# Autodesk Inventor assembly: Battery Pack - Samsung 25R - 2xRows
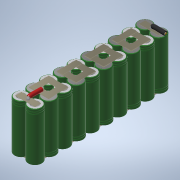
[picture p0: Inventor's stored thumbnail of the model, 180x180]
Saved by Autodesk Inventor 2020.1 (Build 241239000, 239)
## iProperties
Created: 2019-07-13
Part Number: Battery Pack - Samsung 25R - 2xRows
Document SubType Name: Assembly
Designer: Petar
Author: Petar
## Documents named in this file (5)
- D:\OMG\E-Board\CAD\Inventor\Electrical Components\Battery Pack\Samsung 25R\Battery Pack - Samsung 25R - 2xRows.iam
- D:\OMG\E-Board\CAD\Inventor\Electrical Components\Battery Pack\Samsung 25R\Battery Cell - Samsung.ipt
- D:\OMG\E-Board\CAD\Inventor\Electrical Components\Battery Pack\Samsung 25R\Nickel Strip.ipt
- D:\OMG\E-Board\CAD\Inventor\Electrical Components\Battery Pack\Samsung 25R\Solder (Plus).ipt
- D:\OMG\E-Board\CAD\Inventor\Electrical Components\Battery Pack\Samsung 25R\Solder (Minus).ipt
## Components (60 placed, 4 different names)
1. Battery Cell - Samsung:1 — Flush:1, Tangent:1, Flush:2, Flush:5, Flush:6, Tangent:3, Mate:6, Tangent:20, Tangent:22
2. Battery Cell - Samsung:2 — Flush:1, Tangent:1, Flush:2, Tangent:21
3. Battery Cell - Samsung:3 — Flush:5, Flush:6, Tangent:3, Flush:13, Tangent:7, Flush:14
4. Battery Cell - Samsung:4
5. Battery Cell - Samsung:5 — Flush:13, Tangent:7, Flush:14
6. Battery Cell - Samsung:6
7. Battery Cell - Samsung:7 — Flush:29, Tangent:15, Flush:30
8. Battery Cell - Samsung:8
9. Battery Cell - Samsung:9 — Flush:29, Tangent:15, Flush:30
10. Battery Cell - Samsung:10
11. Battery Cell - Samsung:11
12. Battery Cell - Samsung:12
13. Battery Cell - Samsung:13
14. Battery Cell - Samsung:14
15. Battery Cell - Samsung:15 — Flush:37, Tangent:19, Flush:38
16. Battery Cell - Samsung:16
17. Battery Cell - Samsung:17 — Flush:37, Tangent:19, Flush:38
18. Battery Cell - Samsung:18
19. Battery Cell - Samsung:19
20. Battery Cell - Samsung:20
21. Solder (Plus):1 — Flush:43, Rigid:1
22. Solder (Minus):1 — Rigid:2
23. Nickel Strip:1 — Flush:43, Rigid:1
24. Nickel Strip:2 — Mate:5, Mate:6, Flush:39, Flush:40
25. Nickel Strip:3 — Mate:7, Flush:41, Flush:42
26. Nickel Strip:4
27. Nickel Strip:5
28. Nickel Strip:6
29. Nickel Strip:7
30. Nickel Strip:8
31. Nickel Strip:9
32. Nickel Strip:10
33. Nickel Strip:11
34. Nickel Strip:12
35. Nickel Strip:13
36. Nickel Strip:14
37. Nickel Strip:15
38. Nickel Strip:16
39. Nickel Strip:17
40. Nickel Strip:18
41. Nickel Strip:19 — Rigid:2
42. Nickel Strip:20
43. Nickel Strip:21 — Mate:5, Flush:39, Flush:40
44. Nickel Strip:22
45. Nickel Strip:23
46. Nickel Strip:24
47. Nickel Strip:25 — Angle:1
48. Nickel Strip:26 — Angle:3
49. Nickel Strip:27 — Symmetry:1
50. Nickel Strip:28
51. Nickel Strip:29
52. Nickel Strip:30 — Angle:2
53. Nickel Strip:31 — Mate:7, Flush:41, Flush:42
54. Nickel Strip:32 — Symmetry:1
55. Nickel Strip:33
56. Nickel Strip:34
57. Nickel Strip:35
58. Nickel Strip:36
59. Nickel Strip:37
60. Nickel Strip:38
## Component patterns: (20 elements, first: Nickel Strip:1), (10 elements, first: Nickel Strip:21), (8 elements, first: Nickel Strip:31)
## Relationships (74: Flush 43, Tangent 22, Mate 3, Angle 3, WeldJoint 2, Symmetry 1)
- Flush:1: Battery Cell - Samsung:1 ↔ Battery Cell - Samsung:2
- Tangent:1: Battery Cell - Samsung:1 ↔ Battery Cell - Samsung:2
- Flush:2: Battery Cell - Samsung:1 ↔ Battery Cell - Samsung:2
- [Flush]: Battery Cell - Samsung:3 ↔ Battery Cell - Samsung:4
- [Tangent]: Battery Cell - Samsung:3 ↔ Battery Cell - Samsung:4
- [Flush]: Battery Cell - Samsung:3 ↔ Battery Cell - Samsung:4
- Flush:5: Battery Cell - Samsung:1 ↔ Battery Cell - Samsung:3
- Flush:6: Battery Cell - Samsung:1 ↔ Battery Cell - Samsung:3
- Tangent:3: Battery Cell - Samsung:1 ↔ Battery Cell - Samsung:3
- [Flush]: Battery Cell - Samsung:5 ↔ Battery Cell - Samsung:6
- [Tangent]: Battery Cell - Samsung:5 ↔ Battery Cell - Samsung:6
- [Flush]: Battery Cell - Samsung:5 ↔ Battery Cell - Samsung:6
- [Flush]: Battery Cell - Samsung:7 ↔ Battery Cell - Samsung:8
- [Tangent]: Battery Cell - Samsung:7 ↔ Battery Cell - Samsung:8
- [Flush]: Battery Cell - Samsung:7 ↔ Battery Cell - Samsung:8
- [Flush]: Battery Cell - Samsung:5 ↔ Battery Cell - Samsung:7
- [Flush]: Battery Cell - Samsung:5 ↔ Battery Cell - Samsung:7
- [Tangent]: Battery Cell - Samsung:5 ↔ Battery Cell - Samsung:7
- Flush:13: Battery Cell - Samsung:3 ↔ Battery Cell - Samsung:5
- Tangent:7: Battery Cell - Samsung:3 ↔ Battery Cell - Samsung:5
- Flush:14: Battery Cell - Samsung:3 ↔ Battery Cell - Samsung:5
- [Flush]: Battery Cell - Samsung:9 ↔ Battery Cell - Samsung:10
- [Tangent]: Battery Cell - Samsung:9 ↔ Battery Cell - Samsung:10
- [Flush]: Battery Cell - Samsung:9 ↔ Battery Cell - Samsung:10
- [Flush]: Battery Cell - Samsung:11 ↔ Battery Cell - Samsung:12
- [Tangent]: Battery Cell - Samsung:11 ↔ Battery Cell - Samsung:12
- [Flush]: Battery Cell - Samsung:11 ↔ Battery Cell - Samsung:12
- [Flush]: Battery Cell - Samsung:9 ↔ Battery Cell - Samsung:11
- [Flush]: Battery Cell - Samsung:9 ↔ Battery Cell - Samsung:11
- [Tangent]: Battery Cell - Samsung:9 ↔ Battery Cell - Samsung:11
- [Flush]: Battery Cell - Samsung:13 ↔ Battery Cell - Samsung:14
- [Tangent]: Battery Cell - Samsung:13 ↔ Battery Cell - Samsung:14
- [Flush]: Battery Cell - Samsung:13 ↔ Battery Cell - Samsung:14
- [Flush]: Battery Cell - Samsung:15 ↔ Battery Cell - Samsung:16
- [Tangent]: Battery Cell - Samsung:15 ↔ Battery Cell - Samsung:16
- [Flush]: Battery Cell - Samsung:15 ↔ Battery Cell - Samsung:16
- [Flush]: Battery Cell - Samsung:13 ↔ Battery Cell - Samsung:15
- [Flush]: Battery Cell - Samsung:13 ↔ Battery Cell - Samsung:15
- [Tangent]: Battery Cell - Samsung:13 ↔ Battery Cell - Samsung:15
- [Flush]: Battery Cell - Samsung:11 ↔ Battery Cell - Samsung:13
- [Tangent]: Battery Cell - Samsung:11 ↔ Battery Cell - Samsung:13
- [Flush]: Battery Cell - Samsung:11 ↔ Battery Cell - Samsung:13
- Flush:29: Battery Cell - Samsung:7 ↔ Battery Cell - Samsung:9
- Tangent:15: Battery Cell - Samsung:7 ↔ Battery Cell - Samsung:9
- Flush:30: Battery Cell - Samsung:7 ↔ Battery Cell - Samsung:9
- [Flush]: Battery Cell - Samsung:17 ↔ Battery Cell - Samsung:18
- [Tangent]: Battery Cell - Samsung:17 ↔ Battery Cell - Samsung:18
- [Flush]: Battery Cell - Samsung:17 ↔ Battery Cell - Samsung:18
- [Flush]: Battery Cell - Samsung:19 ↔ Battery Cell - Samsung:20
- [Tangent]: Battery Cell - Samsung:19 ↔ Battery Cell - Samsung:20
- [Flush]: Battery Cell - Samsung:19 ↔ Battery Cell - Samsung:20
- [Flush]: Battery Cell - Samsung:17 ↔ Battery Cell - Samsung:19
- [Flush]: Battery Cell - Samsung:17 ↔ Battery Cell - Samsung:19
- [Tangent]: Battery Cell - Samsung:17 ↔ Battery Cell - Samsung:19
- Flush:37: Battery Cell - Samsung:15 ↔ Battery Cell - Samsung:17
- Tangent:19: Battery Cell - Samsung:15 ↔ Battery Cell - Samsung:17
- Flush:38: Battery Cell - Samsung:15 ↔ Battery Cell - Samsung:17
- Mate:5: Nickel Strip:2 ↔ Nickel Strip:21
- Mate:6: Battery Cell - Samsung:1 ↔ Nickel Strip:2
- Flush:39 (0.165 mm): Nickel Strip:2 ↔ Nickel Strip:21
- Flush:40: Nickel Strip:2 ↔ Nickel Strip:21
- Mate:7: Nickel Strip:3 ↔ Nickel Strip:31
- Flush:41: Nickel Strip:3 ↔ Nickel Strip:31
- Flush:42 (0.165 mm): Nickel Strip:3 ↔ Nickel Strip:31
- Symmetry:1: Nickel Strip:27 ↔ Nickel Strip:32
- Angle:1 (0 deg): Nickel Strip:25
- Tangent:20: Battery Cell - Samsung:1
- Angle:2 (0 deg): Nickel Strip:30
- Tangent:21: Battery Cell - Samsung:2
- Angle:3 (0 deg): Nickel Strip:26
- Tangent:22: Battery Cell - Samsung:1
- Flush:43: Solder (Plus):1 ↔ Nickel Strip:1
- Rigid:1 [WeldJoint]: Solder (Plus):1 ↔ Nickel Strip:1
- Rigid:2 [WeldJoint]: Solder (Minus):1 ↔ Nickel Strip:19
## Named parameters: d3_d1 = 0 mm, d4_d2 = 0 mm, d5_d0 = 0 mm, d9_d1 = 0 mm, d10_d2 = 0 mm, d11_d3_d1 = 0 mm, d12_d4_d2 = 0 mm, d13_d5_d0 = 0 mm, d14_d6 = 0 mm, d15_d7 = 0 mm, d16_d8 = 0 mm, d17_d0 = 0 mm, d21_d18 = 0 mm, d22_d19 = 0 mm, d23_d20 = 0 mm, d24_d1 = 0 mm, d25_d2 = 0 mm, d26_d3_d1 = 0 mm, d27_d4_d2 = 0 mm, d28_d5_d0 = 0 mm, d29_d6 = 0 mm, d30_d7 = 0 mm, d31_d8 = 0 mm, d32_d9_d1 = 0 mm, d33_d10_d2 = 0 mm, d34_d11_d3_d1 = 0 mm, d35_d12_d4_d2 = 0 mm, d36_d13_d5_d0 = 0 mm, d37_d14_d6 = 0 mm, d38_d15_d7 = 0 mm, d39_d16_d8 = 0 mm, d40_d17_d0 = 0 mm, d41_d0 = 0 mm, d45_d32_d9_d1 = 0 mm, d46_d33_d10_d2 = 0 mm, d47_d34_d11_d3_d1 = 0 mm, d48_d35_d12_d4_d2 = 0 mm, d49_d36_d13_d5_d0 = 0 mm, d50_d37_d14_d6 = 0 mm, d51_d38_d15_d7 = 0 mm, d52_d39_d16_d8 = 0 mm, d53_d40_d17_d0 = 0 mm
